# Autodesk Inventor assembly: 2 Sensores
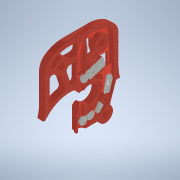
[picture p0: Inventor's stored thumbnail of the model, 180x180]
Saved by Autodesk Inventor 2021 (Build 250183000, 183)
## iProperties
Created: 2021-08-27
Part Number: 2 Sensores
Document SubType Name: Assembly
Designer: Diego.labarca
Author: Diego.labarca
## Documents named in this file (5)
- E:\Dropbox\Inventor\Impresora 3D\Arreglos Impresora\2 Sensores.iam
- E:\Dropbox\Inventor\Impresora 3D\Arreglos Impresora\Brazo Sensor.ipt
- E:\Dropbox\Inventor\Impresora 3D\Arreglos Impresora\Sensores.ipt
- E:\Dropbox\Inventor\Impresora 3D\Arreglos Impresora\Ball 4mm.ipt
- E:\Dropbox\Inventor\Impresora 3D\Arreglos Impresora\Iman 5x3.ipt
## Components (8 placed, 4 different names)
1. Brazo Sensor:1 — Insertar:2
2. Sensores:1 — Coincidencia:1, Coincidencia:2, Coincidencia:5, Insertar:2, Coincidencia:6, Coincidencia:7
3. Ball 4mm:1 — Coincidencia:1, Coincidencia:2, Coincidencia:3, Nivelación:1, Coincidencia:5
4. Ball 4mm:2 — Coincidencia:3, Nivelación:1
5. Ball 4mm:3 — Tangente:1, Coincidencia:6
6. Iman 5x3:1 — Tangente:1, Coincidencia:7, Nivelación:2, Coincidencia:8
7. Iman 5x3:2 — Nivelación:2, Coincidencia:8, Coincidencia:9, Nivelación:3
8. Iman 5x3:3 — Coincidencia:9, Nivelación:3
## Relationships (13: Mate 8, Flush 3, Insert 1, Tangent 1)
- Coincidencia:1 [Mate]: Sensores:1 ↔ Ball 4mm:1
- Coincidencia:2 [Mate] (1 mm): Sensores:1 ↔ Ball 4mm:1
- Coincidencia:3 [Mate]: Ball 4mm:1 ↔ Ball 4mm:2
- Nivelación:1 [Flush] (4 mm): Ball 4mm:1 ↔ Ball 4mm:2
- Coincidencia:5 [Mate] (-4 mm): Sensores:1 ↔ Ball 4mm:1
- Insertar:2: Brazo Sensor:1 ↔ Sensores:1
- Tangente:1: Ball 4mm:3 ↔ Iman 5x3:1
- Coincidencia:6 [Mate]: Sensores:1 ↔ Ball 4mm:3
- Coincidencia:7 [Mate]: Sensores:1 ↔ Iman 5x3:1
- Nivelación:2 [Flush] (-3 mm): Iman 5x3:1 ↔ Iman 5x3:2
- Coincidencia:8 [Mate]: Iman 5x3:1 ↔ Iman 5x3:2
- Coincidencia:9 [Mate]: Iman 5x3:2 ↔ Iman 5x3:3
- Nivelación:3 [Flush] (3 mm): Iman 5x3:2 ↔ Iman 5x3:3
